# Autodesk Inventor assembly: Hopper Idler assy
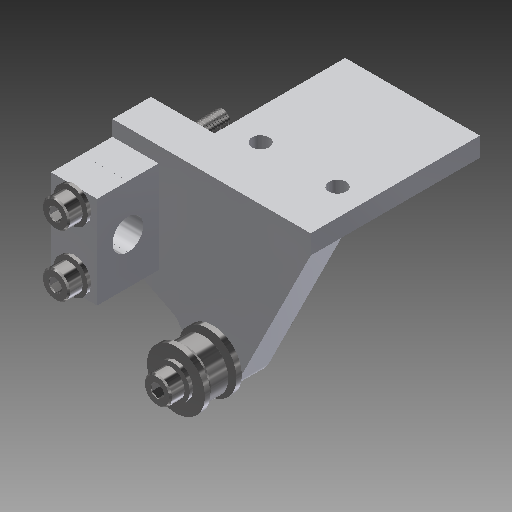
[picture p0: Inventor's stored thumbnail of the model, 512x512]
Saved by Autodesk Inventor 2018 (Build 220112000, 112)
## iProperties
Created: 2017-09-21
Part Number: Hopper Idler assy
Document SubType Name: Assembly
Designer: Gabriel Smolnycki
Author: Gabriel Smolnycki
## Documents named in this file (9)
- E:\planb\mechanics\Subassemblies\Hopper Idler assy.iam
- E:\planb\mechanics\Hopper\Hopper Idler.ipt
- E:\planb\mechanics\Hopper\Hopper Smooth Rod Clamp.ipt
- E:\planb\mechanics\Hardware\M4x40 SS SHCS.ipt
- E:\planb\mechanics\Hardware\M4 SS Washer.ipt
- E:\planb\mechanics\Hardware\M4 SS Locknut.ipt
- E:\planb\mechanics\Hardware\M4x30 SS SHCS.ipt
- E:\planb\mechanics\Hardware\M5 SS Fender Washer.ipt
- E:\planb\mechanics\Hardware\4x13 SS Ball Bearing (7804K103).ipt
## Components (17 placed, 8 different names)
1. Hopper Idler:1 — Insert:1, Insert:2, Insert:17, Insert:18
2. Hopper Smooth Rod Clamp:1 — Insert:1, Insert:2, Insert:3, Insert:4
3. Hopper Smooth Rod Clamp:2 — Insert:3, Insert:4, Insert:5, Insert:6
4. M4x40 SS SHCS:1 — Insert:7
5. M4x40 SS SHCS:2 — Insert:8
6. M4 SS Washer:1 — Insert:6, Insert:7
7. M4 SS Washer:2 — Insert:5, Insert:8
8. M4x30 SS SHCS:1 — Insert:10
9. M4 SS Washer:3 — Insert:10, Insert:11
10. M4 SS Washer:4 — Insert:12, Insert:13
11. M4 SS Washer:5 — Insert:14, Insert:15
12. M4 SS Washer:6 — Insert:16, Insert:17
13. M4 SS Washer:7 — Insert:18, Insert:19
14. M4 SS Locknut:2 — Insert:19
15. M5 SS Fender Washer:1 — Insert:11, Insert:12
16. M5 SS Fender Washer:2 — Insert:15, Insert:16
17. 4x13 SS Ball Bearing (7804K103):1 — Insert:13, Insert:14
## Relationships (18: Insert 18)
- Insert:1: Hopper Idler:1 ↔ Hopper Smooth Rod Clamp:1
- Insert:2: Hopper Idler:1 ↔ Hopper Smooth Rod Clamp:1
- Insert:3: Hopper Smooth Rod Clamp:1 ↔ Hopper Smooth Rod Clamp:2
- Insert:4: Hopper Smooth Rod Clamp:1 ↔ Hopper Smooth Rod Clamp:2
- Insert:5: Hopper Smooth Rod Clamp:2 ↔ M4 SS Washer:2
- Insert:6: Hopper Smooth Rod Clamp:2 ↔ M4 SS Washer:1
- Insert:7: M4x40 SS SHCS:1 ↔ M4 SS Washer:1
- Insert:8: M4x40 SS SHCS:2 ↔ M4 SS Washer:2
- Insert:10: M4x30 SS SHCS:1 ↔ M4 SS Washer:3
- Insert:11: M4 SS Washer:3 ↔ M5 SS Fender Washer:1
- Insert:12: M4 SS Washer:4 ↔ M5 SS Fender Washer:1
- Insert:13: M4 SS Washer:4 ↔ 4x13 SS Ball Bearing (7804K103):1
- Insert:14: M4 SS Washer:5 ↔ 4x13 SS Ball Bearing (7804K103):1
- Insert:15: M4 SS Washer:5 ↔ M5 SS Fender Washer:2
- Insert:16: M4 SS Washer:6 ↔ M5 SS Fender Washer:2
- Insert:17: Hopper Idler:1 ↔ M4 SS Washer:6
- Insert:18: Hopper Idler:1 ↔ M4 SS Washer:7
- Insert:19: M4 SS Washer:7 ↔ M4 SS Locknut:2
